# Autodesk Inventor assembly: Beamerscope_r3
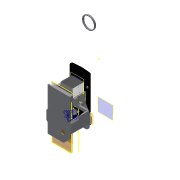
[picture p0: Inventor's stored thumbnail of the model, 180x180]
Saved by Autodesk Inventor 2016 (Build 200138000, 138)
## iProperties
Created: 2016-11-22
Part Number: Beamerscope_r3
Material: Generisch
Document SubType Name: Assembly
Designer: Bene
Author: Bene
## Documents named in this file (5)
- C:\Users\diederichbenedict\Documents\Inventor\Beamerscope_r4\Beamerscope_r3.iam
- C:\Users\diederichbenedict\Documents\Inventor\Beamerscope_r4\Bare_Projector.iam
- C:\Users\diederichbenedict\Documents\Inventor\Beamerscope_r4\Nexus 5.ipt
- C:\Users\diederichbenedict\Documents\Inventor\Beamerscope_r4\02_Coolingfan.ipt
- C:\Users\diederichbenedict\Documents\Inventor\Beamerscope_r4\Mutter.ipt
## Components (4 placed, 4 different names)
1. Bare_Projector:1 [sub-assembly] — Winkel:1, Einfügen:1
2. Nexus 5:1 — Winkel:1, Einfügen:1
3. 02_Coolingfan:1
4. Mutter:1
## Relationships (2: Angle 1, Insert 1)
- Winkel:1 [Angle] (0 deg): Bare_Projector:1 ↔ Nexus 5:1
- Einfügen:1 [Insert] (12 mm): Bare_Projector:1 ↔ Nexus 5:1
